# Autodesk Inventor assembly: DEC_haz
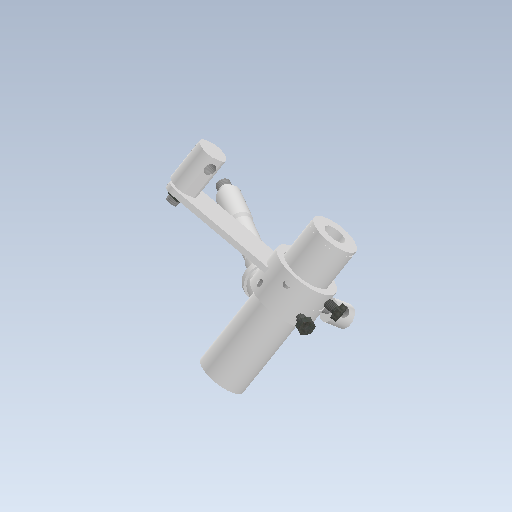
[picture p0: Inventor's stored thumbnail of the model, 512x512]
Saved by Autodesk Inventor 2021 (Build 250183000, 183)
## iProperties
Created: 2023-12-03
Part Number: DEC_haz
Document SubType Name: Assembly
Designer: vtoth
Author: vtoth
## Documents named in this file (10)
- C:\Users\ZenBook\OneDrive - Budapesti Műszaki és Gazdaságtudományi Egyetem\5_felev\CAD\hf2_v2\DEC_haz.iam
- C:\Users\ZenBook\OneDrive - Budapesti Műszaki és Gazdaságtudományi Egyetem\5_felev\CAD\hf2_v2\dec_veg.ipt
- C:\Users\ZenBook\OneDrive - Budapesti Műszaki és Gazdaságtudományi Egyetem\5_felev\CAD\hf2_v2\dec_haz_1.ipt
- C:\Users\ZenBook\OneDrive - Budapesti Műszaki és Gazdaságtudományi Egyetem\5_felev\CAD\hf2_v2\dec_alatet.ipt
- C:\Users\ZenBook\OneDrive - Budapesti Műszaki és Gazdaságtudományi Egyetem\5_felev\CAD\hf2_v2\dec_rogzito.ipt
- C:\Users\ZenBook\OneDrive - Budapesti Műszaki és Gazdaságtudományi Egyetem\5_felev\CAD\hf2_v2\dec_anya.ipt
- C:\Users\ZenBook\OneDrive - Budapesti Műszaki és Gazdaságtudományi Egyetem\5_felev\CAD\hf2_v2\dec_kar.ipt
- C:\Users\ZenBook\OneDrive - Budapesti Műszaki és Gazdaságtudományi Egyetem\5_felev\CAD\hf2_v2\dec_anya2.ipt
- C:\Users\ZenBook\OneDrive - Budapesti Műszaki és Gazdaságtudományi Egyetem\Dokumentumok\Inventor\Content Center Files\R2021\en-US\ISO 4018\ISO 4018 - M8 x 16.ipt
- C:\Users\ZenBook\OneDrive - Budapesti Műszaki és Gazdaságtudományi Egyetem\5_felev\CAD\hf2_v2\ContentCenter\en-US\ISO 4036(2)\ISO 4036 - M10(2).ipt
## Components (11 placed, 9 different names)
1. dec_veg:1 — Insert:1
2. dec_haz_1:1 — Insert:1, Mate:2, Insert:2, Mate:4, Tangent:1, Tangent:2, Tangent:3
3. dec_alatet:1 — Insert:2
4. dec_rogzito:1 — Mate:2, Mate:3, Mate:6, Mate:7, Angle:1, Angle:2
5. dec_anya:1 — Mate:3
6. dec_kar:1 — Insert:3, Mate:4, Mate:5, Angle:3, Insert:4
7. dec_anya2:1 — Insert:3
8. ISO 4018 M8 x 16:1 — Mate:6, Tangent:2, Angle:1
9. ISO 4018 M8 x 16:2 — Mate:7, Tangent:1, Angle:2
10. ISO 4018 M8 x 16:3 — Mate:5, Tangent:3, Angle:3
11. ISO 4036 M10:1 — Insert:4
## Relationships (16: Mate 6, Insert 4, Tangent 3, Angle 3)
- Insert:1: dec_veg:1 ↔ dec_haz_1:1
- Mate:2: dec_haz_1:1 ↔ dec_rogzito:1
- Insert:2: dec_haz_1:1 ↔ dec_alatet:1
- Mate:3: dec_rogzito:1 ↔ dec_anya:1
- Insert:3: dec_kar:1 ↔ dec_anya2:1
- Mate:4: dec_haz_1:1 ↔ dec_kar:1
- Mate:5: dec_kar:1 ↔ ISO 4018 M8 x 16:3
- Mate:6: dec_rogzito:1 ↔ ISO 4018 M8 x 16:1
- Mate:7: dec_rogzito:1 ↔ ISO 4018 M8 x 16:2
- Tangent:1: dec_haz_1:1 ↔ ISO 4018 M8 x 16:2
- Tangent:2: dec_haz_1:1 ↔ ISO 4018 M8 x 16:1
- Tangent:3: dec_haz_1:1 ↔ ISO 4018 M8 x 16:3
- Angle:1 (0 deg): dec_rogzito:1 ↔ ISO 4018 M8 x 16:1
- Angle:2 (0 deg): dec_rogzito:1 ↔ ISO 4018 M8 x 16:2
- Angle:3 (0 deg): dec_kar:1 ↔ ISO 4018 M8 x 16:3
- Insert:4: dec_kar:1 ↔ ISO 4036 M10:1
